# Autodesk Inventor assembly: Drawer
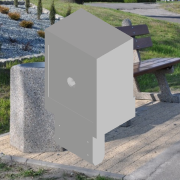
[picture p0: Inventor's stored thumbnail of the model, 180x180]
Saved by Autodesk Inventor 2021 (Build 250183000, 183)
## iProperties
Created: 2025-11-29
Part Number: Drawer
Document SubType Name: Assembly
Designer: huber
Sending System: Autodesk Inventor 2026
Preprocessor: ST-DEVELOPER v20.1
Title: Drawer.stp
Author: Miki
## Documents named in this file (6)
- C:\Users\huber\OneDrive\Pulpit\hackaton BHL\BHL 2025\Drawer.iam
- C:\Users\huber\OneDrive\Pulpit\hackaton BHL\BHL 2025\Ultrasonic sensor.ipt
- C:\Users\huber\OneDrive\Pulpit\hackaton BHL\BHL 2025\Szuflada.ipt
- C:\Users\huber\OneDrive\Pulpit\hackaton BHL\BHL 2025\sensorBox.ipt
- C:\Users\huber\OneDrive\Pulpit\hackaton BHL\BHL 2025\canMount.ipt
- C:\Users\huber\OneDrive\Pulpit\hackaton BHL\BHL 2025\plytka.ipt
## Components (5 placed, 5 different names)
1. Ultrasonic sensor:1 — Mate:3, Mate:4, Mate:5
2. Szuflada:1 — Mate:1, Mate:2, Mate:3, Mate:4, Mate:5, Mate:6
3. sensorBox:1 — Mate:1, Mate:2, Mate:6, Flush:1, Mate:7
4. canMount:1 — Insert:1, Mate:7
5. plytka:1 — Flush:1, Insert:1
## Relationships (9: Mate 7, Flush 1, Insert 1)
- Mate:1: Szuflada:1 ↔ sensorBox:1
- Mate:2 (0.5 mm): Szuflada:1 ↔ sensorBox:1
- Mate:3: Ultrasonic sensor:1 ↔ Szuflada:1
- Mate:4: Ultrasonic sensor:1 ↔ Szuflada:1
- Mate:5: Ultrasonic sensor:1 ↔ Szuflada:1
- Mate:6: Szuflada:1 ↔ sensorBox:1
- Flush:1: sensorBox:1 ↔ plytka:1
- Insert:1: canMount:1 ↔ plytka:1
- Mate:7: sensorBox:1 ↔ canMount:1
